# Autodesk Inventor assembly: mountstestfit
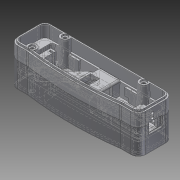
[picture p0: Inventor's stored thumbnail of the model, 180x180]
Saved by Autodesk Inventor 2014 SP1 (Build 180222100, 222)
## iProperties
Created: 2014-04-06
Part Number: mountstestfit
Document SubType Name: Assembly
Designer: Tyler
Author: Tyler
## Documents named in this file (3)
- C:\Users\Tyler\Documents\housing\mountstestfit.iam
- C:\Users\Tyler\Documents\housing\case_rear.ipt
- C:\Users\Tyler\Documents\housing\case_front.ipt
## Components (2 placed, 2 different names)
1. case_front:1 — Flush:1, Flush:2, Mate:1
2. case_rear:1 — Flush:1, Flush:2, Mate:1
## Relationships (3: Flush 2, Mate 1)
- Flush:1: case_front:1 ↔ case_rear:1
- Flush:2: case_front:1 ↔ case_rear:1
- Mate:1: case_front:1 ↔ case_rear:1
